# Autodesk Inventor assembly: Assy_upper_arm
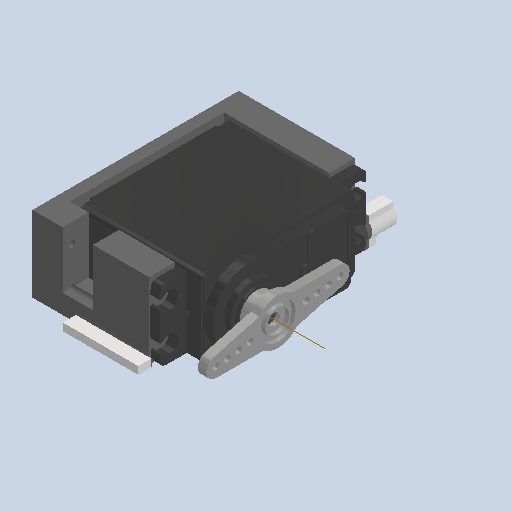
[picture p0: Inventor's stored thumbnail of the model, 512x512]
Saved by Autodesk Inventor 2024.1 (Build 281209000, 209)
## iProperties
Created: 2025-03-03
Part Number: Assy_upper_arm
Document SubType Name: Assembly
Designer: hibik
Author: hibik
## Documents named in this file (5)
- C:\Users\hibik\Documents\Robomech\RESCUE\ORCA\hard\arm\Assy_upper_arm.iam
- C:\Users\hibik\Documents\Robomech\RESCUE\ORCA\hard\std_parts\FS5103B.ipt
- C:\Users\hibik\Documents\Robomech\RESCUE\ORCA\hard\std_parts\feetech_servohone.ipt
- C:\Users\hibik\Documents\Robomech\RESCUE\ORCA\hard\std_parts\bearing_6_10_3.ipt
- C:\Users\hibik\Documents\Robomech\RESCUE\ORCA\hard\arm\upper_arm_base_with_connector.iam
## Components (4 placed, 4 different names)
1. FS5103B:1 — 挿入:1, メイト:6, 角度:2
2. feetech_servohone:1 — 挿入:1, メイト:4
3. bearing_6_10_3:1 — 挿入:2
4. upper_arm_base_with_connector:1 [sub-assembly] — フラッシュ:1, メイト:5, 角度:1, 挿入:2, メイト:6
## Relationships (8: Mate 3, Insert 2, Angle 2, Flush 1)
- 挿入:1 [Insert]: FS5103B:1 ↔ feetech_servohone:1
- メイト:4 [Mate]: feetech_servohone:1
- フラッシュ:1 [Flush]: upper_arm_base_with_connector:1
- メイト:5 [Mate]: upper_arm_base_with_connector:1
- 角度:1 [Angle] (180 deg): upper_arm_base_with_connector:1
- 挿入:2 [Insert]: bearing_6_10_3:1 ↔ upper_arm_base_with_connector:1
- メイト:6 [Mate]: FS5103B:1 ↔ upper_arm_base_with_connector:1
- 角度:2 [Angle] (0 deg): FS5103B:1
